# Autodesk Inventor assembly: top_cover
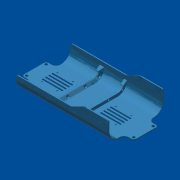
[picture p0: Inventor's stored thumbnail of the model, 180x180]
Saved by Autodesk Inventor 2019 (Build 230136000, 136)
## iProperties
Created: 2020-10-03
Part Number: top_cover
Document SubType Name: Assembly
Designer: ewdia
Author: ewdia
## Documents named in this file (4)
- C:\Users\ewdia\Downloads\balam_assembly parts\top_cover\top_cover.iam
- C:\Users\ewdia\Downloads\balam_assembly parts\top_cover\Imported Components\TopCover_1\TopCover_1.ipt
- C:\Users\ewdia\Downloads\balam_assembly parts\top_cover\Imported Components\TopCoverSpacer\TopCoverSpacer.ipt
- C:\Users\ewdia\Downloads\balam_assembly parts\top_cover\Imported Components\TopCover_2\TopCover_2.ipt
## Components (3 placed, 3 different names)
1. TopCover_1:1 — Rigid:1
2. TopCoverSpacer:1 — Rigid:1, Rigid:2
3. TopCover_2:1 — Rigid:2
## Relationships (2: WeldJoint 2)
- Rigid:1 [WeldJoint]: TopCover_1:1 ↔ TopCoverSpacer:1
- Rigid:2 [WeldJoint]: TopCoverSpacer:1 ↔ TopCover_2:1
